# Autodesk Inventor assembly: Model
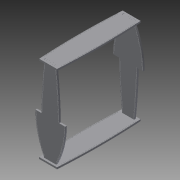
[picture p0: Inventor's stored thumbnail of the model, 180x180]
Saved by Autodesk Inventor 2015 (Build 190159000, 159)
## iProperties
Created: 2016-08-21
Part Number: Model
Document SubType Name: Assembly
Designer: Alex Bello
Author: Alex Bello
## Documents named in this file (3)
- C:\Users\Alex Bello\Documents\GitHub\Linear Construction No 1\Model.iam
- C:\Users\Alex Bello\Documents\GitHub\Linear Construction No 1\Parts\Side.ipt
- C:\Users\Alex Bello\Documents\GitHub\Linear Construction No 1\Parts\Top.ipt
## Components (4 placed, 2 different names)
1. Side:1 — Flush:3, Mate:5, Mate:6
2. Top:1 — Flush:2, Mate:3, Mate:4, Flush:3, Mate:6
3. Side:2 — Flush:1, Mate:1, Mate:2, Flush:2, Mate:3, Mate:4
4. Top:2 — Flush:1, Mate:1, Mate:2, Mate:5
## Relationships (9: Mate 6, Flush 3)
- Flush:1: Side:2 ↔ Top:2
- Mate:1: Side:2 ↔ Top:2
- Mate:2: Side:2 ↔ Top:2
- Flush:2: Top:1 ↔ Side:2
- Mate:3: Top:1 ↔ Side:2
- Mate:4: Top:1 ↔ Side:2
- Flush:3: Side:1 ↔ Top:1
- Mate:5: Side:1 ↔ Top:2
- Mate:6: Side:1 ↔ Top:1
